# Autodesk Inventor assembly: A2017_T2_03
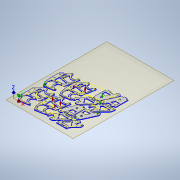
[picture p0: Inventor's stored thumbnail of the model, 180x180]
Saved by Autodesk Inventor 2020 (Build 240168000, 168)
## iProperties
Created: 2021-08-27
Part Number: A2017_T2_03
Document SubType Name: Assembly
Designer: Masato
Author: Masato
## Documents named in this file (5)
- C:\Users\naoki\Documents\Inventor\CitBrains\git_clone\SUSTAINA_ver1_0\A_T4_T2\SUSTAINA-OP\Cam\A2017_T2_03.iam
- C:\Users\naoki\Documents\Inventor\CitBrains\git_clone\SUSTAINA_ver1_0\A_T4_T2\SUSTAINA-OP\Cam\DisposableBoard.ipt
- C:\Users\naoki\Documents\Inventor\CitBrains\git_clone\SUSTAINA_ver1_0\A_T4_T2\SUSTAINA-OP\LowerBody\Knee\Knee_side_frame.ipt
- C:\Users\naoki\Documents\Inventor\CitBrains\git_clone\SUSTAINA_ver1_0\A_T4_T2\SUSTAINA-OP\LowerBody\Leg_joit\Leg_joint_pitch_frame.ipt
- C:\Users\naoki\Documents\Inventor\CitBrains\git_clone\SUSTAINA_ver1_0\A_T4_T2\SUSTAINA-OP\UpperBody\Arm\Shoulder_side_frame.ipt
## Components (13 placed, 4 different names)
1. DisposableBoard:1 — メイト:2, メイト:1, フラッシュ:1, フラッシュ:2, 正接:1, フラッシュ:3, メイト:4, メイト:7, メイト:8, メイト:9, メイト:10, フラッシュ:4, フラッシュ:5, メイト:19, メイト:20, メイト:21, メイト:22
2. Leg_joint_pitch_frame:1 — メイト:10, メイト:14, メイト:15, 正接:2, フラッシュ:6, メイト:24
3. Leg_joint_pitch_frame:2 — メイト:9, メイト:13, メイト:14, フラッシュ:6, メイト:23
4. Shoulder_side_frame:2 — メイト:7, フラッシュ:4, メイト:11, メイト:13
5. Shoulder_side_frame:1 — メイト:8, メイト:11, フラッシュ:5, メイト:15
6. Shoulder_side_frame:3 — メイト:17, メイト:18, メイト:20, メイト:24, 正接:4
7. Shoulder_side_frame:4 — メイト:18, メイト:19, メイト:23, メイト:25
8. Leg_joint_pitch_frame:3 — 正接:3, メイト:16, メイト:17, メイト:21
9. Leg_joint_pitch_frame:4 — 正接:3, メイト:16, メイト:22, メイト:25
10. Knee_side_frame:1 — 正接:1, フラッシュ:3, メイト:4
11. Knee_side_frame:3
12. Knee_side_frame:4 — 正接:2
13. Knee_side_frame:5 — 正接:4
## Component patterns: (4 elements, first: Knee_side_frame:1)
## Relationships (31: Mate 21, Flush 6, Tangent 4)
- メイト:2 [Mate]: DisposableBoard:1
- メイト:1 [Mate]: DisposableBoard:1
- フラッシュ:1 [Flush]: DisposableBoard:1
- フラッシュ:2 [Flush]: DisposableBoard:1
- 正接:1 [Tangent] (2.5 mm): DisposableBoard:1 ↔ Knee_side_frame:1
- フラッシュ:3 [Flush] (2 mm): DisposableBoard:1 ↔ Knee_side_frame:1
- メイト:4 [Mate]: DisposableBoard:1 ↔ Knee_side_frame:1
- メイト:7 [Mate]: DisposableBoard:1 ↔ Shoulder_side_frame:2
- メイト:8 [Mate]: DisposableBoard:1 ↔ Shoulder_side_frame:1
- メイト:9 [Mate]: DisposableBoard:1 ↔ Leg_joint_pitch_frame:2
- メイト:10 [Mate]: DisposableBoard:1 ↔ Leg_joint_pitch_frame:1
- フラッシュ:4 [Flush] (2 mm): DisposableBoard:1 ↔ Shoulder_side_frame:2
- メイト:11 [Mate] (2.5 mm): Shoulder_side_frame:2 ↔ Shoulder_side_frame:1
- メイト:13 [Mate] (2.5 mm): Leg_joint_pitch_frame:2 ↔ Shoulder_side_frame:2
- メイト:14 [Mate] (2.5 mm): Leg_joint_pitch_frame:1 ↔ Leg_joint_pitch_frame:2
- フラッシュ:5 [Flush] (2 mm): DisposableBoard:1 ↔ Shoulder_side_frame:1
- メイト:15 [Mate] (2.5 mm): Leg_joint_pitch_frame:1 ↔ Shoulder_side_frame:1
- 正接:2 [Tangent] (2.5 mm): Leg_joint_pitch_frame:1 ↔ Knee_side_frame:4
- フラッシュ:6 [Flush]: Leg_joint_pitch_frame:1 ↔ Leg_joint_pitch_frame:2
- 正接:3 [Tangent]: Leg_joint_pitch_frame:3 ↔ Leg_joint_pitch_frame:4
- メイト:16 [Mate] (2.5 mm): Leg_joint_pitch_frame:3 ↔ Leg_joint_pitch_frame:4
- メイト:17 [Mate] (2.5 mm): Shoulder_side_frame:3 ↔ Leg_joint_pitch_frame:3
- メイト:18 [Mate] (2.5 mm): Shoulder_side_frame:3 ↔ Shoulder_side_frame:4
- メイト:19 [Mate]: DisposableBoard:1 ↔ Shoulder_side_frame:4
- メイト:20 [Mate]: DisposableBoard:1 ↔ Shoulder_side_frame:3
- メイト:21 [Mate]: DisposableBoard:1 ↔ Leg_joint_pitch_frame:3
- メイト:22 [Mate]: DisposableBoard:1 ↔ Leg_joint_pitch_frame:4
- メイト:23 [Mate] (2.5 mm): Leg_joint_pitch_frame:2 ↔ Shoulder_side_frame:4
- メイト:24 [Mate] (2.5 mm): Leg_joint_pitch_frame:1 ↔ Shoulder_side_frame:3
- 正接:4 [Tangent] (2.5 mm): Shoulder_side_frame:3 ↔ Knee_side_frame:5
- メイト:25 [Mate] (2.5 mm): Shoulder_side_frame:4 ↔ Leg_joint_pitch_frame:4
